# Autodesk Inventor assembly: Custom Cover Assembly
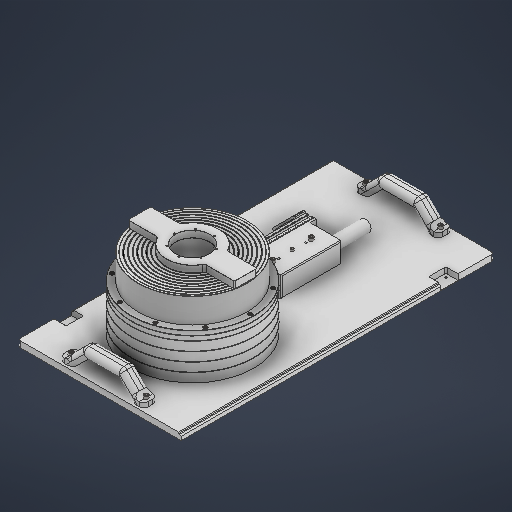
[picture p0: Inventor's stored thumbnail of the model, 512x512]
Saved by Autodesk Inventor 2025 (Build 290162000, 162)
## iProperties
Created: 2024-04-26
Part Number: Custom Cover Assembly
Document SubType Name: Assembly
Designer: Thienan Hoang
Author: Thienan Hoang
## Documents named in this file (22)
- C:\Users\mayhe\OneDrive\Documents\In-situ-monitoring-of-powder-bed-fusion-additive-manufacturing\system_development\Orichalcum\v0.1\Hardware_design\custom-cover\Custom Cover Full Assembly.iam
- C:\Users\mayhe\OneDrive\Documents\In-situ-monitoring-of-powder-bed-fusion-additive-manufacturing\system_development\Orichalcum\v0.1\Hardware_design\custom-cover\cover\Updated Cover.ipt
- C:\Users\mayhe\OneDrive\Documents\In-situ-monitoring-of-powder-bed-fusion-additive-manufacturing\system_development\Orichalcum\v0.1\Hardware_design\laser-vibrometer\Updated Laser Scanner.ipt
- C:\Users\mayhe\OneDrive\Documents\In-situ-monitoring-of-powder-bed-fusion-additive-manufacturing\system_development\Orichalcum\v0.1\Hardware_design\laser-vibrometer\Updated Laser Bracket.ipt
- C:\Users\mayhe\OneDrive\Documents\In-situ-monitoring-of-powder-bed-fusion-additive-manufacturing\system_development\Orichalcum\v0.1\Hardware_design\custom-cover\8020-parts\25-4136.ipt
- C:\Users\mayhe\OneDrive\Documents\In-situ-monitoring-of-powder-bed-fusion-additive-manufacturing\system_development\Orichalcum\v0.1\Hardware_design\custom-cover\8020-parts\11-4310.ipt
- C:\Users\mayhe\OneDrive\Documents\In-situ-monitoring-of-powder-bed-fusion-additive-manufacturing\system_development\Orichalcum\v0.1\Hardware_design\custom-cover\8020-parts\20-2020-160-CL.ipt
- C:\Users\mayhe\OneDrive\Documents\In-situ-monitoring-of-powder-bed-fusion-additive-manufacturing\system_development\Orichalcum\v0.1\Hardware_design\custom-cover\8020-parts\14159_m.ipt
- C:\Users\mayhe\OneDrive\Documents\In-situ-monitoring-of-powder-bed-fusion-additive-manufacturing\system_development\Orichalcum\v0.1\Hardware_design\galvo-scanner\GVS102.iam
- C:\Users\mayhe\OneDrive\Documents\In-situ-monitoring-of-powder-bed-fusion-additive-manufacturing\system_development\Orichalcum\v0.1\Hardware_design\custom-cover\8020-parts\20-2020-200-CL.ipt
- C:\Users\mayhe\OneDrive\Documents\In-situ-monitoring-of-powder-bed-fusion-additive-manufacturing\system_development\Orichalcum\v0.1\Hardware_design\custom-cover\8020-parts\25-1964.ipt
- C:\Users\mayhe\OneDrive\Documents\In-situ-monitoring-of-powder-bed-fusion-additive-manufacturing\system_development\Orichalcum\v0.1\Hardware_design\custom-cover\cylinder-parts\final-parts\Cylinder Spacer Bottom.ipt
- C:\Users\mayhe\OneDrive\Documents\In-situ-monitoring-of-powder-bed-fusion-additive-manufacturing\system_development\Orichalcum\v0.1\Hardware_design\custom-cover\cylinder-parts\final-parts\Cylinder Spacer Top.ipt
- C:\Users\mayhe\OneDrive\Documents\In-situ-monitoring-of-powder-bed-fusion-additive-manufacturing\system_development\Orichalcum\v0.1\Hardware_design\custom-cover\cylinder-parts\final-parts\Cylinder Slidey Bit.iam
- C:\Users\mayhe\OneDrive\Documents\In-situ-monitoring-of-powder-bed-fusion-additive-manufacturing\system_development\Orichalcum\v0.1\Hardware_design\custom-cover\cylinder-parts\final-parts\Cylinder Spacer 25mm.ipt
- C:\Users\mayhe\OneDrive\Documents\In-situ-monitoring-of-powder-bed-fusion-additive-manufacturing\system_development\Orichalcum\v0.1\Hardware_design\custom-cover\cylinder-parts\cylinder-segments\Head Thing.ipt
- C:\Users\mayhe\OneDrive\Documents\In-situ-monitoring-of-powder-bed-fusion-additive-manufacturing\system_development\Orichalcum\v0.1\Hardware_design\custom-cover\cylinder-parts\final-parts\Cylinder Bottom.ipt
- C:\Users\mayhe\OneDrive\Documents\In-situ-monitoring-of-powder-bed-fusion-additive-manufacturing\system_development\Orichalcum\v0.1\Hardware_design\custom-cover\cover\Handles.ipt
- C:\Users\mayhe\OneDrive\Documents\In-situ-monitoring-of-powder-bed-fusion-additive-manufacturing\system_development\Orichalcum\v0.1\Hardware_design\custom-cover\8020-parts\ANSI B18.3.1M - M2x0.4 x 20(1).ipt
- C:\Users\mayhe\OneDrive\Documents\In-situ-monitoring-of-powder-bed-fusion-additive-manufacturing\system_development\Orichalcum\v0.1\Hardware_design\custom-cover\8020-parts\ANSI B18.3.1M - M6x1 x 20(1).ipt
- C:\Users\mayhe\OneDrive\Documents\In-situ-monitoring-of-powder-bed-fusion-additive-manufacturing\system_development\Orichalcum\v0.1\Hardware_design\custom-cover\8020-parts\ANSI B18.3.1M - M4x0.7 x 6(1).ipt
- C:\Users\mayhe\OneDrive\Documents\In-situ-monitoring-of-powder-bed-fusion-additive-manufacturing\system_development\Orichalcum\v0.1\Hardware_design\custom-cover\8020-parts\ANSI B18.3.1M - M5x0.8 x 100(1).ipt
## Components (62 placed, 21 different names)
1. Updated Cover:1 — Mate:15, Mate:17, Mate:18, Mate:19, Mate:20, Mate:32, Mate:33, Flush:5, Mate:48, Mate:82, Mate:86, Mate:98, Mate:106, Mate:107, Mate:108, Mate:109
2. 11-4310:10 — Mate:125, Mate:130
3. 11-4310:11 — Mate:126, Mate:132
4. 11-4310:12 — Mate:127, Mate:136
5. 11-4310:13 — Mate:128, Mate:134
6. GVS102:1 [sub-assembly] — Mate:66, Mate:67, Angle:2
7. 20-2020-200-CL:1 — Mate:69, Flush:8, Mate:85, Angle:2, Mate:122, Mate:123, Mate:124
8. 25-1964:1 — Mate:66, Mate:67, Mate:69, Flush:8, Mate:85
9. Updated Laser Bracket:1 — Flush:9, Mate:83, Rotational:15, Mate:86, Insert:22, Insert:23, Insert:24, Mate:125, Mate:126, Mate:127, Mate:128
10. Updated Laser Scanner:1 — Rotational:15
11. Head Thing:1 — Mate:110, Mate:111, Insert:11, Insert:12, Insert:13, Insert:14, Insert:15, Insert:16, Insert:17
12. Cylinder Bottom:1 — Mate:98, Mate:99, Mate:100
13. Cylinder Spacer Bottom:1 — Mate:99, Mate:100, Mate:101, Mate:102, Mate:122, Mate:123, Mate:124
14. Cylinder Spacer Top:1 — Mate:101, Mate:102, Mate:103, Mate:104
15. Cylinder Spacer 25mm:1 — Mate:103, Mate:104, Mate:105, Rotational:16
16. Cylinder Slidey Bit:1 [sub-assembly] — Mate:105, Rotational:16, Mate:110, Mate:111, Mate:112, Mate:113, Mate:114, Mate:115, Mate:116, Mate:117, Mate:118, Mate:119, Mate:120, Mate:121
17. Handles:1 — Mate:108, Mate:109, Insert:18, Insert:19
18. Handles:2 — Mate:106, Mate:107, Insert:20, Insert:21
19. 14159_m:5 — Mate:131, Mate:132
20. 14159_m:6 — Mate:135, Mate:136
21. 14159_m:7 — Mate:129, Mate:130
22. 14159_m:8 — Mate:133, Mate:134
23. 25-4136:1 — Mate:5, Mate:6, Mate:9, Mate:10, Flush:1, Flush:2, Mate:15, Mate:17, Mate:18, Rotational:2, Rigid:1
24. 20-2020-160-CL:1 — Flush:1, Mate:11, Mate:12, Flush:9, Mate:83, Mate:129, Mate:133
25. 11-4310:1 — Mate:5, Mate:8
26. 11-4310:2 — Mate:6, Mate:7
27. 14159_m:1 — Mate:8, Mate:10, Mate:13, Mate:14
28. 14159_m:2 — Mate:7, Mate:9, Mate:11, Mate:12
29. 20-2020-160-CL:2 — Flush:2, Mate:13, Mate:14, Mate:56, Mate:131, Mate:135
30. 11-4310:3 — Rotational:2
31. 11-4310:4 — Rigid:1
32. 25-4136:3 — Mate:19, Mate:20, Rotational:3, Rotational:4, Rotational:5, Rotational:6, Mate:23, Mate:32, Mate:33, Mate:82
33. 11-4310:6 — Rotational:3
34. 11-4310:7 — Rotational:4
35. 11-4310:8 — Rotational:5, Mate:21
36. 11-4310:9 — Rotational:6, Mate:22
37. 14159_m:3 — Mate:22, Mate:56
38. 14159_m:4 — Mate:21, Mate:23
39. Forged Socket Head Cap Screw - Metric M2x0.4 x 20:1 — Insert:11
40. Forged Socket Head Cap Screw - Metric M2x0.4 x 20:2 — Insert:12
41. Forged Socket Head Cap Screw - Metric M2x0.4 x 20:3 — Insert:13
42. Forged Socket Head Cap Screw - Metric M2x0.4 x 20:4 — Insert:14
43. Forged Socket Head Cap Screw - Metric M2x0.4 x 20:5 — Insert:15
44. Forged Socket Head Cap Screw - Metric M2x0.4 x 20:6 — Insert:16
45. Forged Socket Head Cap Screw - Metric M2x0.4 x 20:7 — Insert:17
46. Forged Socket Head Cap Screw - Metric M6x1 x 20:1 — Insert:18
47. Forged Socket Head Cap Screw - Metric M6x1 x 20:2 — Insert:19
48. Forged Socket Head Cap Screw - Metric M6x1 x 20:3 — Insert:20
49. Forged Socket Head Cap Screw - Metric M6x1 x 20:4 — Insert:21
50. Forged Socket Head Cap Screw - Metric M6x1 x 20:5 — Insert:22
51. Forged Socket Head Cap Screw - Metric M6x1 x 20:6 — Insert:23
52. Forged Socket Head Cap Screw - Metric M4x0.7 x 6:1 — Insert:24
53. Forged Socket Head Cap Screw - Metric M5x0.8 x 100:1 — Mate:112
54. Forged Socket Head Cap Screw - Metric M5x0.8 x 100:3 — Mate:118
55. Forged Socket Head Cap Screw - Metric M5x0.8 x 100:4 — Mate:115
56. Forged Socket Head Cap Screw - Metric M5x0.8 x 100:5 — Mate:113
57. Forged Socket Head Cap Screw - Metric M5x0.8 x 100:6 — Mate:120
58. Forged Socket Head Cap Screw - Metric M5x0.8 x 100:7 — Mate:121
59. Forged Socket Head Cap Screw - Metric M5x0.8 x 100:8 — Mate:119
60. Forged Socket Head Cap Screw - Metric M5x0.8 x 100:9 — Mate:117
61. Forged Socket Head Cap Screw - Metric M5x0.8 x 100:10 — Mate:116
62. Forged Socket Head Cap Screw - Metric M5x0.8 x 100:11 — Mate:114
## Relationships (97: Mate 68, Insert 14, RevoluteJoint 7, Flush 6, WeldJoint 1, Angle 1)
- Mate:5: 25-4136:1 ↔ 11-4310:1
- Mate:6: 25-4136:1 ↔ 11-4310:2
- Mate:7: 11-4310:2 ↔ 14159_m:2
- Mate:8: 11-4310:1 ↔ 14159_m:1
- Mate:9 (1.5 mm): 25-4136:1 ↔ 14159_m:2
- Mate:10 (1.5 mm): 25-4136:1 ↔ 14159_m:1
- Flush:1: 25-4136:1 ↔ 20-2020-160-CL:1
- Flush:2: 25-4136:1 ↔ 20-2020-160-CL:2
- Mate:11: 20-2020-160-CL:1 ↔ 14159_m:2
- Mate:12 (1.5 mm): 20-2020-160-CL:1 ↔ 14159_m:2
- Mate:13: 14159_m:1 ↔ 20-2020-160-CL:2
- Mate:14 (1.45 mm): 14159_m:1 ↔ 20-2020-160-CL:2
- Mate:15: Updated Cover:1 ↔ 25-4136:1
- Mate:17: Updated Cover:1 ↔ 25-4136:1
- Mate:18: Updated Cover:1 ↔ 25-4136:1
- Rotational:2 [RevoluteJoint]: 25-4136:1 ↔ 11-4310:3
- Rigid:1 [WeldJoint]: 25-4136:1 ↔ 11-4310:4
- Mate:19: Updated Cover:1 ↔ 25-4136:3
- Mate:20: Updated Cover:1 ↔ 25-4136:3
- Rotational:3 [RevoluteJoint]: 25-4136:3 ↔ 11-4310:6
- Rotational:4 [RevoluteJoint]: 25-4136:3 ↔ 11-4310:7
- Rotational:5 [RevoluteJoint]: 25-4136:3 ↔ 11-4310:8
- Rotational:6 [RevoluteJoint]: 25-4136:3 ↔ 11-4310:9
- Mate:21: 11-4310:8 ↔ 14159_m:4
- Mate:22: 11-4310:9 ↔ 14159_m:3
- Mate:23 (1.5 mm): 25-4136:3 ↔ 14159_m:4
- Mate:32: Updated Cover:1 ↔ 25-4136:3
- Mate:33: Updated Cover:1 ↔ 25-4136:3
- Flush:5 (180 mm): Updated Cover:1
- Mate:48: Updated Cover:1
- Flush:6 (38 mm)
- Mate:56: 20-2020-160-CL:2 ↔ 14159_m:3
- Mate:66: GVS102:1 ↔ 25-1964:1
- Mate:67 (1.5 mm): GVS102:1 ↔ 25-1964:1
- Mate:69 (0.52 mm): 20-2020-200-CL:1 ↔ 25-1964:1
- Flush:8 (34 mm): 20-2020-200-CL:1 ↔ 25-1964:1
- Mate:82: Updated Cover:1 ↔ 25-4136:3
- Flush:9: Updated Laser Bracket:1 ↔ 20-2020-160-CL:1
- Mate:83: Updated Laser Bracket:1 ↔ 20-2020-160-CL:1
- Mate:85: 20-2020-200-CL:1 ↔ 25-1964:1
- Rotational:15 [RevoluteJoint]: Updated Laser Bracket:1 ↔ Updated Laser Scanner:1
- Mate:86 (1.5 mm): Updated Cover:1 ↔ Updated Laser Bracket:1
- Angle:2 (0 deg): GVS102:1 ↔ 20-2020-200-CL:1
- Mate:98: Updated Cover:1 ↔ Cylinder Bottom:1
- Mate:99: Cylinder Bottom:1 ↔ Cylinder Spacer Bottom:1
- Mate:100: Cylinder Bottom:1 ↔ Cylinder Spacer Bottom:1
- Mate:101: Cylinder Spacer Bottom:1 ↔ Cylinder Spacer Top:1
- Mate:102: Cylinder Spacer Bottom:1 ↔ Cylinder Spacer Top:1
- Mate:103: Cylinder Spacer Top:1 ↔ Cylinder Spacer 25mm:1
- Mate:104: Cylinder Spacer Top:1 ↔ Cylinder Spacer 25mm:1
- Mate:105: Cylinder Spacer 25mm:1 ↔ Cylinder Slidey Bit:1
- Rotational:16 [RevoluteJoint]: Cylinder Spacer 25mm:1 ↔ Cylinder Slidey Bit:1
- Mate:106: Updated Cover:1 ↔ Handles:2
- Mate:107: Updated Cover:1 ↔ Handles:2
- Mate:108: Updated Cover:1 ↔ Handles:1
- Mate:109: Updated Cover:1 ↔ Handles:1
- Mate:110: Head Thing:1 ↔ Cylinder Slidey Bit:1
- Mate:111: Head Thing:1 ↔ Cylinder Slidey Bit:1
- Insert:11: Head Thing:1 ↔ Forged Socket Head Cap Screw - Metric M2x0.4 x 20:1
- Insert:12: Head Thing:1 ↔ Forged Socket Head Cap Screw - Metric M2x0.4 x 20:2
- Insert:13: Head Thing:1 ↔ Forged Socket Head Cap Screw - Metric M2x0.4 x 20:3
- Insert:14: Head Thing:1 ↔ Forged Socket Head Cap Screw - Metric M2x0.4 x 20:4
- Insert:15: Head Thing:1 ↔ Forged Socket Head Cap Screw - Metric M2x0.4 x 20:5
- Insert:16: Head Thing:1 ↔ Forged Socket Head Cap Screw - Metric M2x0.4 x 20:6
- Insert:17: Head Thing:1 ↔ Forged Socket Head Cap Screw - Metric M2x0.4 x 20:7
- Insert:18: Handles:1 ↔ Forged Socket Head Cap Screw - Metric M6x1 x 20:1
- Insert:19: Handles:1 ↔ Forged Socket Head Cap Screw - Metric M6x1 x 20:2
- Insert:20: Handles:2 ↔ Forged Socket Head Cap Screw - Metric M6x1 x 20:3
- Insert:21: Handles:2 ↔ Forged Socket Head Cap Screw - Metric M6x1 x 20:4
- Insert:22: Updated Laser Bracket:1 ↔ Forged Socket Head Cap Screw - Metric M6x1 x 20:5
- Insert:23: Updated Laser Bracket:1 ↔ Forged Socket Head Cap Screw - Metric M6x1 x 20:6
- Insert:24: Updated Laser Bracket:1 ↔ Forged Socket Head Cap Screw - Metric M4x0.7 x 6:1
- Mate:112: Cylinder Slidey Bit:1 ↔ Forged Socket Head Cap Screw - Metric M5x0.8 x 100:1
- Mate:113: Cylinder Slidey Bit:1 ↔ Forged Socket Head Cap Screw - Metric M5x0.8 x 100:5
- Mate:114: Cylinder Slidey Bit:1 ↔ Forged Socket Head Cap Screw - Metric M5x0.8 x 100:11
- Mate:115: Cylinder Slidey Bit:1 ↔ Forged Socket Head Cap Screw - Metric M5x0.8 x 100:4
- Mate:116: Cylinder Slidey Bit:1 ↔ Forged Socket Head Cap Screw - Metric M5x0.8 x 100:10
- Mate:117: Cylinder Slidey Bit:1 ↔ Forged Socket Head Cap Screw - Metric M5x0.8 x 100:9
- Mate:118: Cylinder Slidey Bit:1 ↔ Forged Socket Head Cap Screw - Metric M5x0.8 x 100:3
- Mate:119: Cylinder Slidey Bit:1 ↔ Forged Socket Head Cap Screw - Metric M5x0.8 x 100:8
- Mate:120: Cylinder Slidey Bit:1 ↔ Forged Socket Head Cap Screw - Metric M5x0.8 x 100:6
- Mate:121: Cylinder Slidey Bit:1 ↔ Forged Socket Head Cap Screw - Metric M5x0.8 x 100:7
- Mate:122: 20-2020-200-CL:1 ↔ Cylinder Spacer Bottom:1
- Mate:123: 20-2020-200-CL:1 ↔ Cylinder Spacer Bottom:1
- Mate:124: 20-2020-200-CL:1 ↔ Cylinder Spacer Bottom:1
- Mate:125: 11-4310:10 ↔ Updated Laser Bracket:1
- Mate:126: 11-4310:11 ↔ Updated Laser Bracket:1
- Mate:127: 11-4310:12 ↔ Updated Laser Bracket:1
- Mate:128: 11-4310:13 ↔ Updated Laser Bracket:1
- Mate:129: 14159_m:7 ↔ 20-2020-160-CL:1
- Mate:130: 11-4310:10 ↔ 14159_m:7
- Mate:131: 14159_m:5 ↔ 20-2020-160-CL:2
- Mate:132: 11-4310:11 ↔ 14159_m:5
- Mate:133: 14159_m:8 ↔ 20-2020-160-CL:1
- Mate:134: 11-4310:13 ↔ 14159_m:8
- Mate:135: 14159_m:6 ↔ 20-2020-160-CL:2
- Mate:136: 11-4310:12 ↔ 14159_m:6
